# Autodesk Inventor assembly: Schreibtisch
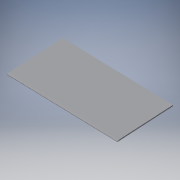
[picture p0: Inventor's stored thumbnail of the model, 180x180]
Saved by Autodesk Inventor 2017 (Build 210142000, 142)
## iProperties
Created: 2017-06-01
Part Number: Schreibtisch
Document SubType Name: Assembly
Designer: Fake
Author: Fake
## Documents named in this file (3)
- C:\Users\Fake\Documents\Inventor\Oli_Grundstück\Schreibtisch.iam
- C:\Users\Fake\Documents\Inventor\Oli_Grundstück\Arbeitsplatte.ipt
- C:\Users\Fake\Documents\Inventor\Oli_Grundstück\Tischbein.ipt
## Components (2 placed, 2 different names)
1. Arbeitsplatte:1 — Passend:1
2. Tischbein:1
## Relationships (1: Mate 1)
- Passend:1 [Mate]: Arbeitsplatte:1
